# Autodesk Inventor assembly: Assembly_Spiral_XY_MGN7-grooves-MB
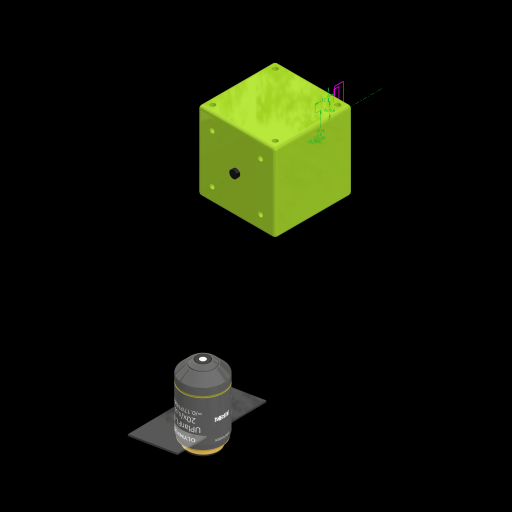
[picture p0: Inventor's stored thumbnail of the model, 512x512]
Saved by Autodesk Inventor 2024 (Build 280153000, 153)
## iProperties
Created: 2023-09-18
Part Number: Assembly_Spiral_XY_MGN7-grooves-MB
Document SubType Name: Assembly
Designer: diederichbenedict
Author: diederichbenedict
## Documents named in this file (8)
- E:\User\Dokumente\#BeneEspressoscope\Assembly_Spiral_XY_MGN7-grooves-MB.iam
- Assembly_Spiral_XY_MGN9.iam
- E:\User\Dokumente\#BeneEspressoscope\00_Sample_Doubleslit.ipt
- E:\User\Dokumente\#BeneEspressoscope\00_Microscope_objective_4x.ipt
- E:\User\Dokumente\#BeneEspressoscope\00_NEMA_17.ipt
- E:\User\Dokumente\#BeneEspressoscope\55_spiralxy_motorplate_nema_mgn9.ipt
- E:\User\Dokumente\#BeneEspressoscope\55_spiralxy_slidemount_MGN9_Nema17_Body.ipt
- E:\User\Dokumente\#BeneEspressoscope\55_spiralxy_spiral-groove.ipt
## Components (7 placed, 6 different names)
1. 00_Sample_Doubleslit:1
2. 00_Microscope_objective_4x:1
3. 00_NEMA_17:1
4. 55_spiralxy_slidemount_MGN9_Nema17_Body:1 — Passend:12, Winkel:3, Passend:13
5. 00_NEMA_17:2 — Passend:12, Winkel:3, Passend:13, Einfügen:7, Winkel:4
6. 55_spiralxy_motorplate_nema_mgn9:1 — Einfügen:7, Winkel:4
7. 55_spiralxy_spiral-groove:1
## Relationships (7: Angle 3, Mate 2, Insert 2)
- Passend:12 [Mate]: 55_spiralxy_slidemount_MGN9_Nema17_Body:1 ↔ 00_NEMA_17:2
- Winkel:3 [Angle] (180 deg): 55_spiralxy_slidemount_MGN9_Nema17_Body:1 ↔ 00_NEMA_17:2
- Passend:13 [Mate]: 55_spiralxy_slidemount_MGN9_Nema17_Body:1 ↔ 00_NEMA_17:2
- Einfügen:7 [Insert]: 00_NEMA_17:2 ↔ 55_spiralxy_motorplate_nema_mgn9:1
- Winkel:4 [Angle] (180 deg): 00_NEMA_17:2 ↔ 55_spiralxy_motorplate_nema_mgn9:1
- [Insert]: 55_spiralxy_motorplate_nema_mgn9:1 ↔ 55_spiralxy_spiral-groove:1
- [Angle] (0 deg): 00_NEMA_17:2 ↔ 55_spiralxy_spiral-groove:1
